# Autodesk Inventor assembly: DRO Case 3
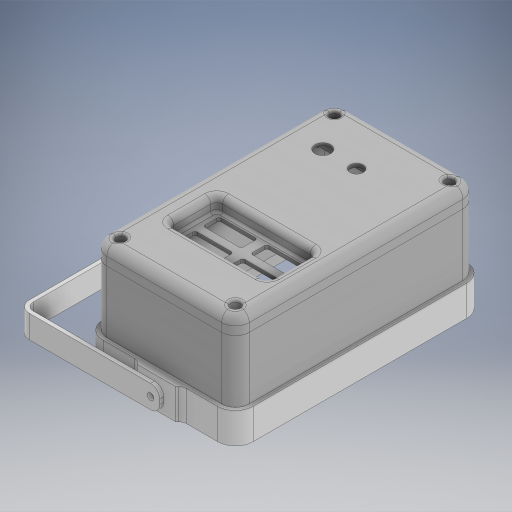
[picture p0: Inventor's stored thumbnail of the model, 512x512]
Saved by Autodesk Inventor 2024 (Build 280153000, 153)
## iProperties
Created: 2024-03-12
Part Number: DRO Case 3
Document SubType Name: Assembly
Designer: AdminForWorker
Title: DRO Case 3 v9
Author: AdminForWorker
## Documents named in this file (10)
- C:\Users\Stefano\Documents\Inventor\drdro\DRO Case 3.iam
- C:\Users\Stefano\Documents\Inventor\drdro\Component1.ipt
- C:\Users\Stefano\Documents\Inventor\drdro\Component4.ipt
- C:\Users\Stefano\Documents\Inventor\drdro\raspberry pi display.iam
- C:\Users\Stefano\Documents\Inventor\drdro\Fascia.ipt
- C:\Users\Stefano\Documents\Inventor\Content Center Files\R2024\en-US\ANSI B18.2.3.5M\ANSI B18.2.3.5M - M5 x 0.8 x 16.ipt
- C:\Users\Stefano\Documents\Inventor\Content Center Files\R2024\en-US\ANSI B18.3.1M(6)\ANSI B18.3.1M - M3x0.5 x 25(1).ipt
- C:\Users\Stefano\Documents\Inventor\Content Center Files\R2024\en-US\ANSI B 18.2.4.1 M(1)\ANSI B 18.2.4.1 M - M3 x 0.5Style 2.ipt
- C:\Users\Stefano\Documents\Inventor\Content Center Files\R2024\en-US\ANSI B18.22 M\ANSI B18.22M - 5 R.ipt
- C:\Users\Stefano\Documents\Inventor\drdro\Pivoting Bracket.ipt
## Components (11 placed, 9 different names)
1. Body — Rotational:1, Mate:1, Flush:1, Flush:2
2. Back Cover
3. raspberry pi display:1 [sub-assembly] — Rotational:1, Mate:1
4. Fascia:1 — Flush:1, Flush:2, Insert:1, Insert:2, Insert:3, Insert:4, Insert:5, Insert:6, Mate:2, Angle:1, Flush:5
5. Hex Bolt - Metric M5 x 0.8 x 16:1 — Insert:1
6. Hex Bolt - Metric M5 x 0.8 x 16:2 — Insert:2
7. Forged Socket Head Cap Screw - Metric M3x0.5 x 25:1 — Insert:3
8. Hex Nut Metric M3 x 0.5:1 — Insert:4
9. Plain Washer (Metric) 5 R:1 — Insert:5
10. Plain Washer (Metric) 5 R:2 — Insert:6
11. Pivoting Bracket:1 — Flush:3, Flush:4, Flush:5
## Relationships (15: Insert 6, Flush 5, Mate 2, RevoluteJoint 1, Angle 1)
- Rotational:1 [RevoluteJoint]: Body ↔ raspberry pi display:1
- Mate:1: Body ↔ raspberry pi display:1
- Flush:1: Body ↔ Fascia:1
- Flush:2: Body ↔ Fascia:1
- Insert:1: Fascia:1 ↔ Hex Bolt - Metric M5 x 0.8 x 16:1
- Insert:2: Fascia:1 ↔ Hex Bolt - Metric M5 x 0.8 x 16:2
- Insert:3: Fascia:1 ↔ Forged Socket Head Cap Screw - Metric M3x0.5 x 25:1
- Insert:4: Fascia:1 ↔ Hex Nut Metric M3 x 0.5:1
- Insert:5: Fascia:1 ↔ Plain Washer (Metric) 5 R:1
- Insert:6: Fascia:1 ↔ Plain Washer (Metric) 5 R:2
- Flush:3: Pivoting Bracket:1
- Mate:2: Fascia:1
- Angle:1 (0 deg): Fascia:1
- Flush:4: Pivoting Bracket:1
- Flush:5: Fascia:1 ↔ Pivoting Bracket:1
